# Autodesk Inventor assembly: Feeder
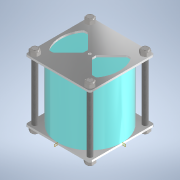
[picture p0: Inventor's stored thumbnail of the model, 180x180]
Saved by Autodesk Inventor 2020.3 (Build 243373000, 373)
## iProperties
Created: 2020-07-23
Part Number: Feeder
Document SubType Name: Assembly
Designer: juanp
Author: juanp
## Documents named in this file (6)
- C:\Users\juanp\Desktop\ROBOCOL\Idea Final NAF\Feeder.iam
- C:\Users\juanp\Desktop\ROBOCOL\Idea Final NAF\Feeder Bottom Plate.ipt
- C:\Users\juanp\Desktop\ROBOCOL\Idea Final NAF\Feeder Rotator.ipt
- C:\Users\juanp\Desktop\ROBOCOL\Idea Final NAF\Feeder Top Plate.ipt
- C:\Users\juanp\Desktop\ROBOCOL\Idea Final NAF\Barra Roscada M5.ipt
- C:\Users\juanp\Desktop\ROBOCOL\Idea Final NAF\Gantry\Inventor\M5 Nylock.ipt
## Components (15 placed, 5 different names)
1. Feeder Bottom Plate:1 — Mate:1, Mate:4, Angle:1, Mate:7, Mate:22, Mate:23, Mate:24
2. Feeder Rotator:1 — Mate:1, Mate:2, Mate:3, Mate:4
3. Feeder Top Plate:1 — Mate:2, Mate:3, Angle:1, Mate:5, Flush:1, Mate:9, Mate:16, Mate:17, Mate:18, Flush:2, Flush:3, Flush:4, Mate:19, Mate:20, Mate:21
4. Barra Roscada M5:1 — Mate:5, Flush:1, Mate:6, Mate:8
5. M5 Nylock:1 — Mate:8, Mate:9
6. M5 Nylock:2 — Mate:6, Mate:7
7. Barra Roscada M5:2 — Mate:17, Flush:4
8. M5 Nylock:3 — Mate:19
9. M5 Nylock:4 — Mate:22
10. Barra Roscada M5:3 — Mate:16, Flush:3
11. M5 Nylock:5 — Mate:20
12. M5 Nylock:6 — Mate:23
13. Barra Roscada M5:4 — Mate:18, Flush:2
14. M5 Nylock:7 — Mate:21
15. M5 Nylock:8 — Mate:24
## Relationships (29: Mate 24, Flush 4, Angle 1)
- Mate:1: Feeder Bottom Plate:1 ↔ Feeder Rotator:1
- Mate:2: Feeder Rotator:1 ↔ Feeder Top Plate:1
- Mate:3: Feeder Rotator:1 ↔ Feeder Top Plate:1
- Mate:4: Feeder Bottom Plate:1 ↔ Feeder Rotator:1
- Angle:1 (90 deg): Feeder Bottom Plate:1 ↔ Feeder Top Plate:1
- Mate:5: Feeder Top Plate:1 ↔ Barra Roscada M5:1
- Flush:1 (-5 mm): Feeder Top Plate:1 ↔ Barra Roscada M5:1
- Mate:6: Barra Roscada M5:1 ↔ M5 Nylock:2
- Mate:7: Feeder Bottom Plate:1 ↔ M5 Nylock:2
- Mate:8: Barra Roscada M5:1 ↔ M5 Nylock:1
- Mate:9: Feeder Top Plate:1 ↔ M5 Nylock:1
- [Mate]: Barra Roscada M5:2 ↔ M5 Nylock:4
- [Mate]: Barra Roscada M5:2 ↔ M5 Nylock:3
- [Mate]: Barra Roscada M5:3 ↔ M5 Nylock:6
- [Mate]: Barra Roscada M5:3 ↔ M5 Nylock:5
- [Mate]: Barra Roscada M5:4 ↔ M5 Nylock:8
- [Mate]: Barra Roscada M5:4 ↔ M5 Nylock:7
- Mate:16: Feeder Top Plate:1 ↔ Barra Roscada M5:3
- Mate:17: Feeder Top Plate:1 ↔ Barra Roscada M5:2
- Mate:18: Feeder Top Plate:1 ↔ Barra Roscada M5:4
- Flush:2 (-5 mm): Feeder Top Plate:1 ↔ Barra Roscada M5:4
- Flush:3 (-5 mm): Feeder Top Plate:1 ↔ Barra Roscada M5:3
- Flush:4 (-5 mm): Feeder Top Plate:1 ↔ Barra Roscada M5:2
- Mate:19: Feeder Top Plate:1 ↔ M5 Nylock:3
- Mate:20: Feeder Top Plate:1 ↔ M5 Nylock:5
- Mate:21: Feeder Top Plate:1 ↔ M5 Nylock:7
- Mate:22: Feeder Bottom Plate:1 ↔ M5 Nylock:4
- Mate:23: Feeder Bottom Plate:1 ↔ M5 Nylock:6
- Mate:24: Feeder Bottom Plate:1 ↔ M5 Nylock:8
## Named parameters: d14_d10 = 0 mm, d15_d12 = 0 mm, d16_d10 = 0 mm, d17_d12 = 0 mm, d18_d10 = 0 mm, d19_d12 = 0 mm
